# Autodesk Inventor assembly: Assembly_cellSTORM_meandric
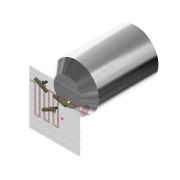
[picture p0: Inventor's stored thumbnail of the model, 180x180]
Saved by Autodesk Inventor 2019.4 (Build 234330000, 330)
## iProperties
Created: 2020-09-02
Part Number: Assembly_cellSTORM_meandric
Document SubType Name: Assembly
Designer: diederichbenedict
Author: diederichbenedict
## Documents named in this file (6)
- C:\Users\diederichbenedict\Dropbox\Dokumente\Promotion\PROJECTS\STORMoChip\GITHUB\CAD\Nanoscopy-on-the-cheap\Workspace\Assembly_cellSTORM_meandric.iam
- C:\Users\diederichbenedict\Dropbox\Dokumente\Promotion\PROJECTS\STORMoChip\GITHUB\CAD\Nanoscopy-on-the-cheap\Workspace\cellSTORM_laserbeam_meander.ipt
- C:\Users\diederichbenedict\Dropbox\Dokumente\Promotion\PROJECTS\STORMoChip\GITHUB\CAD\Nanoscopy-on-the-cheap\Workspace\cellSTORM_laserbeam_meander_chip.ipt
- C:\Users\diederichbenedict\Dropbox\Dokumente\Promotion\PROJECTS\STORMoChip\GITHUB\CAD\Nanoscopy-on-the-cheap\Workspace\Brilliant Krunk.ipt
- C:\Users\diederichbenedict\Dropbox\Dokumente\Promotion\PROJECTS\STORMoChip\GITHUB\CAD\Nanoscopy-on-the-cheap\Workspace\ecoli.ipt
- C:\Users\diederichbenedict\Dropbox\Dokumente\Promotion\PROJECTS\STORMoChip\GITHUB\CAD\Nanoscopy-on-the-cheap\Workspace\objectivelens.ipt
## Components (8 placed, 5 different names)
1. cellSTORM_laserbeam_meander:1 — Flush:1, Tangent:1, Tangent:2, Tangent:3
2. cellSTORM_laserbeam_meander_chip:1 — Flush:1, Flush:2, Flush:3
3. Brilliant Krunk:1 — Tangent:4
4. ecoli:1 — Tangent:1, Tangent:5
5. ecoli:2 — Tangent:3
6. ecoli:3 — Tangent:2, Tangent:4
7. Brilliant Krunk:2 — Tangent:5
8. objectivelens:1 — Flush:2, Flush:3
## Relationships (8: Tangent 5, Flush 3)
- Flush:1: cellSTORM_laserbeam_meander:1 ↔ cellSTORM_laserbeam_meander_chip:1
- Tangent:1: cellSTORM_laserbeam_meander:1 ↔ ecoli:1
- Tangent:2: cellSTORM_laserbeam_meander:1 ↔ ecoli:3
- Tangent:3: cellSTORM_laserbeam_meander:1 ↔ ecoli:2
- Tangent:4: Brilliant Krunk:1 ↔ ecoli:3
- Tangent:5: ecoli:1 ↔ Brilliant Krunk:2
- Flush:2: cellSTORM_laserbeam_meander_chip:1 ↔ objectivelens:1
- Flush:3 (43 mm): cellSTORM_laserbeam_meander_chip:1 ↔ objectivelens:1
